# Autodesk Inventor assembly: MaleHeaderPin_1x5
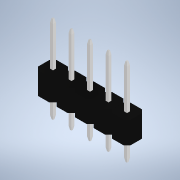
[picture p0: Inventor's stored thumbnail of the model, 180x180]
Saved by Autodesk Inventor 2020 (Build 240168000, 168)
## iProperties
Created: 2020-01-06
Part Number: MaleHeaderPin_1x5
Document SubType Name: Assembly
Designer: ermoz
Author: ermoz
## Documents named in this file (2)
- D:\Moje Wyczyny\Liceum\VLOat INTvators\Moje projekty\Processor Project (kontynuacja)\Drugie podejście\Electric Elements\MaleHeaderPin_1x5.iam
- D:\Moje Wyczyny\Liceum\VLOat INTvators\Moje projekty\Processor Project (kontynuacja)\Drugie podejście\Electric Elements\MaleHeaderPin.ipt
## Components (5 placed, 1 different names)
1. MaleHeaderPin:1 — Flush:1, Flush:8, Flush:9, Mate:1, Mate:2
2. MaleHeaderPin:2 — Flush:1, Flush:2, Flush:8, Mate:1
3. MaleHeaderPin:3 — Flush:2, Flush:3, Flush:9, Flush:10, Mate:2, Mate:3
4. MaleHeaderPin:4 — Flush:3, Flush:4, Flush:10, Flush:11, Mate:3, Mate:4
5. MaleHeaderPin:5 — Flush:4, Flush:11, Mate:4
## Relationships (12: Flush 8, Mate 4)
- Flush:1: MaleHeaderPin:1 ↔ MaleHeaderPin:2
- Flush:2: MaleHeaderPin:2 ↔ MaleHeaderPin:3
- Flush:3: MaleHeaderPin:3 ↔ MaleHeaderPin:4
- Flush:4: MaleHeaderPin:4 ↔ MaleHeaderPin:5
- Flush:8: MaleHeaderPin:1 ↔ MaleHeaderPin:2
- Flush:9: MaleHeaderPin:1 ↔ MaleHeaderPin:3
- Flush:10: MaleHeaderPin:3 ↔ MaleHeaderPin:4
- Flush:11: MaleHeaderPin:4 ↔ MaleHeaderPin:5
- Mate:1: MaleHeaderPin:1 ↔ MaleHeaderPin:2
- Mate:2: MaleHeaderPin:1 ↔ MaleHeaderPin:3
- Mate:3: MaleHeaderPin:3 ↔ MaleHeaderPin:4
- Mate:4: MaleHeaderPin:4 ↔ MaleHeaderPin:5
